# Autodesk Inventor assembly: AssemblyP2
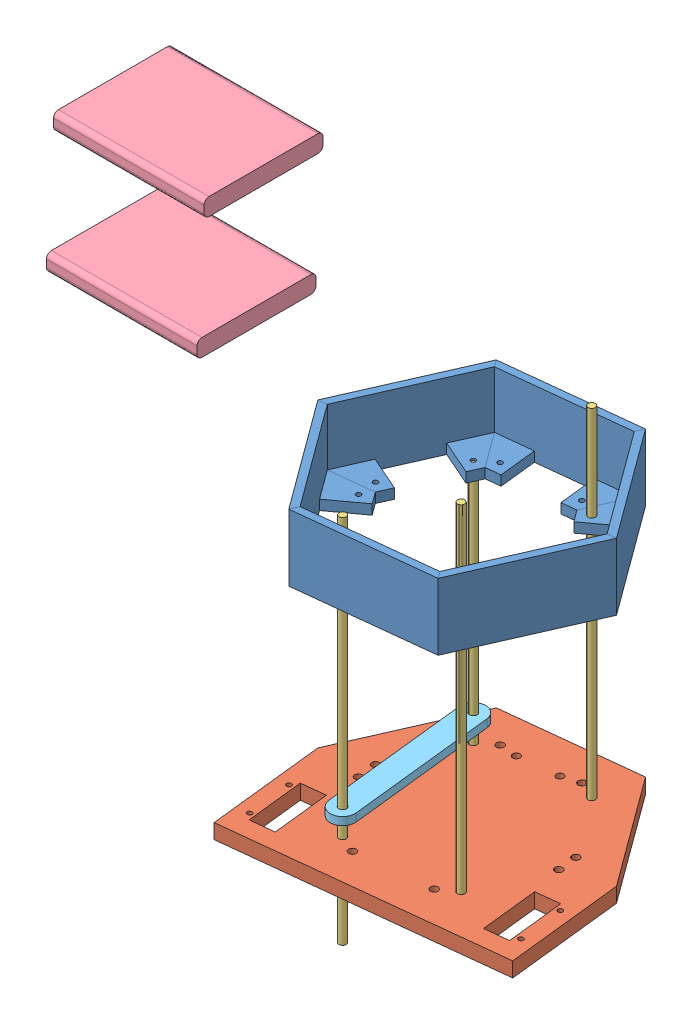
[picture p0: shaded view drawn from the shape stored in the file]
Saved by Autodesk Inventor 2018 (Build 220112000, 112)
## iProperties
Created: 2017-04-19
Part Number: AssemblyP2
Document SubType Name: Assembly
Designer: Pablo
Author: Pablo
## Documents named in this file (6)
- C:\Users\Vidal Villegas\Desktop\mp\AssemblyP2.iam
- C:\Users\Vidal Villegas\Desktop\mp\mp3mp3.ipt
- C:\Users\Vidal Villegas\Downloads\megapr.ipt
- C:\Users\Vidal Villegas\Desktop\mp\tornillo.ipt
- C:\Users\Vidal Villegas\Desktop\mp\portabateria.ipt
- C:\Users\Vidal Villegas\Desktop\mp\lipo.bateria.ipt
## Components (14 placed, 5 different names)
1. mp3mp3:1 — Mate:1, Flush:1, Flush:2, Flush:3, Flush:4, Flush:5, Mate:6, Mate:7, Flush:6
2. mp3mp3:2 — Mate:1, Flush:1, Mate:2, Mate:7, Mate:8
3. mp3mp3:3 — Flush:4, Mate:4, Mate:5, Mate:10
4. mp3mp3:4 — Mate:2, Flush:2, Mate:3, Mate:8, Mate:9
5. mp3mp3:5 — Flush:3, Mate:5, Mate:6, Flush:7, Mate:14
6. mp3mp3:6 — Flush:5, Mate:3, Mate:4, Mate:9, Mate:10
7. megapr:1 — Flush:6, Flush:7, Cylindrical:1, Cylindrical:4, Mate:11, Mate:13, Mate:17, Mate:18
8. tornillo:1 — Mate:13, Mate:14
9. tornillo:2 — Cylindrical:1
10. tornillo:3 — Mate:11
11. tornillo:4 — Cylindrical:4
12. lipo.bateria:1
13. lipo.bateria:2
14. portabateria:1 — Mate:17, Mate:18
## Relationships (24: Mate 15, Flush 7, CylindricalJoint 2)
- Mate:1: mp3mp3:1 ↔ mp3mp3:2
- Flush:1: mp3mp3:1 ↔ mp3mp3:2
- Mate:2: mp3mp3:2 ↔ mp3mp3:4
- Flush:2: mp3mp3:1 ↔ mp3mp3:4
- Flush:3: mp3mp3:1 ↔ mp3mp3:5
- Flush:4: mp3mp3:1 ↔ mp3mp3:3
- Flush:5: mp3mp3:1 ↔ mp3mp3:6
- Mate:3: mp3mp3:4 ↔ mp3mp3:6
- Mate:4: mp3mp3:3 ↔ mp3mp3:6
- Mate:5: mp3mp3:3 ↔ mp3mp3:5
- Mate:6: mp3mp3:1 ↔ mp3mp3:5
- Mate:7: mp3mp3:1 ↔ mp3mp3:2
- Mate:8: mp3mp3:2 ↔ mp3mp3:4
- Mate:9: mp3mp3:4 ↔ mp3mp3:6
- Mate:10: mp3mp3:3 ↔ mp3mp3:6
- Flush:6: mp3mp3:1 ↔ megapr:1
- Flush:7: mp3mp3:5 ↔ megapr:1
- Cylindrical:1: megapr:1 ↔ tornillo:2
- Cylindrical:4: megapr:1 ↔ tornillo:4
- Mate:11: megapr:1 ↔ tornillo:3
- Mate:13: megapr:1 ↔ tornillo:1
- Mate:14: mp3mp3:5 ↔ tornillo:1
- Mate:17 (-33.055 mm): megapr:1 ↔ portabateria:1
- Mate:18: megapr:1 ↔ portabateria:1
